# Autodesk Inventor assembly: main climber
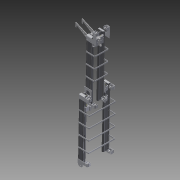
[picture p0: Inventor's stored thumbnail of the model, 180x180]
Saved by Autodesk Inventor 2013 (Build 170138000, 138)
## iProperties
Created: 2013-01-25
Part Number: main climber
Document SubType Name: Assembly
Designer: Arpan
Mass: 7886.47 g
Surface Area: 13806 cm^2
Volume: 3109.24 cm^3
Density: 2.53646 g/cm^3
Author: Arpan
## Documents named in this file (5)
- C:\Users\Arpan\Documents\GitHub\frc2013CAD\Cimber actual\main climber.iam
- C:\Users\Arpan\Documents\GitHub\frc2013CAD\Cimber actual\14 inch shaft.ipt
- C:\Users\Arpan\Documents\GitHub\frc2013CAD\Cimber actual\Inner rails.iam
- C:\Users\Arpan\Documents\GitHub\frc2013CAD\Cimber actual\outer rails.iam
- C:\Users\Arpan\Documents\GitHub\frc2013CAD\Cimber actual\mini pulley assembly.iam
## Components (7 placed, 4 different names)
1. Inner rails:1 [sub-assembly] — Mate:1, Angle:1, Flush:1
2. outer rails:1 [sub-assembly] — Mate:1, Mate:2, Angle:1, Flush:1, Mate:3, Flush:2, Flush:3, Mate:10, Mate:11, Mate:12, Mate:13, Mate:14, Mate:15, Mate:22, Mate:23, Mate:24, Flush:4
3. 14 inch shaft:1 — Mate:2, Flush:4
4. mini pulley assembly:2 [sub-assembly] — Mate:13, Mate:14, Mate:15
5. mini pulley assembly:3 [sub-assembly] — Mate:22, Mate:23, Mate:24
6. mini pulley assembly:5 [sub-assembly] — Mate:3, Flush:2, Flush:3
7. mini pulley assembly:8 [sub-assembly] — Mate:10, Mate:11, Mate:12
## Relationships (17: Mate 12, Flush 4, Angle 1)
- Mate:1: Inner rails:1 ↔ outer rails:1
- Mate:2: outer rails:1 ↔ 14 inch shaft:1
- Angle:1 (180 deg): Inner rails:1 ↔ outer rails:1
- Flush:1 (495.3 mm): Inner rails:1 ↔ outer rails:1
- Mate:3: outer rails:1 ↔ mini pulley assembly:5
- Flush:2: outer rails:1 ↔ mini pulley assembly:5
- Flush:3: outer rails:1 ↔ mini pulley assembly:5
- Mate:10: outer rails:1 ↔ mini pulley assembly:8
- Mate:11: outer rails:1 ↔ mini pulley assembly:8
- Mate:12: outer rails:1 ↔ mini pulley assembly:8
- Mate:13: outer rails:1 ↔ mini pulley assembly:2
- Mate:14: outer rails:1 ↔ mini pulley assembly:2
- Mate:15: outer rails:1 ↔ mini pulley assembly:2
- Mate:22: outer rails:1 ↔ mini pulley assembly:3
- Mate:23: outer rails:1 ↔ mini pulley assembly:3
- Mate:24: outer rails:1 ↔ mini pulley assembly:3
- Flush:4 (-82.8929 mm): outer rails:1 ↔ 14 inch shaft:1
